# Autodesk Inventor assembly: Full Assembly
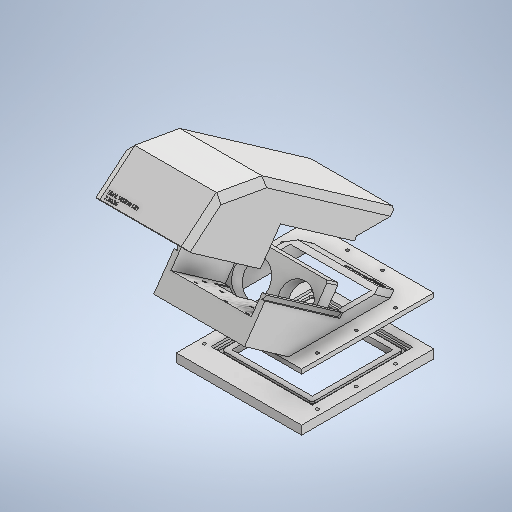
[picture p0: Inventor's stored thumbnail of the model, 512x512]
Saved by Autodesk Inventor 2025.2 (Build 292293000, 293)
## iProperties
Created: 2025-08-13
Part Number: Full Assembly
Document SubType Name: Assembly
Designer: mateo
Author: mateo
## Documents named in this file (4)
- C:\GitHub\In-situ-monitoring-of-powder-bed-fusion-additive-manufacturing\system_development\Damascus\v0.5\Full Assembly.iam
- C:\GitHub\In-situ-monitoring-of-powder-bed-fusion-additive-manufacturing\system_development\Damascus\v0.5\Glass holder.ipt
- C:\GitHub\In-situ-monitoring-of-powder-bed-fusion-additive-manufacturing\system_development\Damascus\v0.5\cameraholderbody v0.5.ipt
- C:\GitHub\In-situ-monitoring-of-powder-bed-fusion-additive-manufacturing\system_development\Damascus\v0.5\cameraholderlid v0.5.ipt
## Components (3 placed, 3 different names)
1. Glass holder:1 — Insert:1
2. cameraholderbody v0.5:1 — Insert:1
3. cameraholderlid v0.5:1
## Relationships (1: Insert 1)
- Insert:1 (50.8 mm): Glass holder:1 ↔ cameraholderbody v0.5:1
